# Autodesk Inventor assembly: spool holder
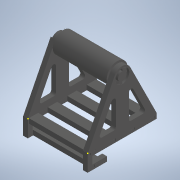
[picture p0: Inventor's stored thumbnail of the model, 180x180]
Saved by Autodesk Inventor 2020.2 (Build 242310000, 310)
## iProperties
Created: 2020-02-09
Part Number: spool holder
Document SubType Name: Assembly
Designer: mulve
Mass: 535.152 g
Surface Area: 1295.84 cm^2
Volume: 411.655 cm^3
Density: 1.3 g/cm^3
Author: mulve
## Documents named in this file (12)
- C:\Users\mulve\github\cad\spool holder\spool holder.iam
- C:\Users\mulve\github\cad\spool holder\spool holder.ipt
- C:\Users\mulve\github\cad\spool holder\spool holder arm.ipt
- C:\Users\mulve\github\cad\spool holder\spool holder span.ipt
- C:\Users\mulve\github\cad\spool holder\spool axle.ipt
- C:\Users\mulve\github\cad\spool holder\spool holder arm side2.ipt
- C:\Users\mulve\github\cad\spool holder\spool holder\AIP\FEA\d58jxclds.fins
- C:\Users\mulve\github\cad\spool holder\spool holder\AIP\FEA\d58jxclds.fsat
- C:\Users\mulve\github\cad\spool holder\spool holder\AIP\FEA\d58jxclds.ftes
- C:\Users\mulve\github\cad\spool holder\spool holder\AIP\FEA\d58jxclds.fwiz
- C:\Users\mulve\github\cad\spool holder\spool holder\AIP\FEA\d58jxclnk.fmsh
- C:\Users\mulve\github\cad\spool holder\spool holder\AIP\FEA\d58jxclnl.fres
## Components (10 placed, 5 different names)
1. spool holder:1 — Mate:4, Mate:5, Flush:1, Mate:6, Mate:7, Flush:2, Mate:8, Mate:9, Flush:3, Mate:10, Mate:11, Flush:4, Mate:12, Mate:13, Flush:5, Mate:18, Flush:8, Mate:19
2. spool holder:2 — Mate:14, Mate:15, Flush:6, Mate:16, Mate:17, Flush:7
3. spool holder arm:1 — Mate:16, Mate:17, Flush:7
4. spool holder span:1 — Mate:4, Mate:5, Flush:1
5. spool holder span:2 — Mate:6, Mate:7, Flush:2, Mate:14, Mate:15, Flush:6
6. spool holder span:3 — Mate:8, Mate:9, Flush:3
7. spool holder span:4 — Mate:10, Mate:11, Flush:4
8. spool holder span:5 — Mate:12, Mate:13, Flush:5
9. spool axle:1
10. spool holder arm side2:1 — Mate:18, Flush:8, Mate:19
## Relationships (24: Mate 16, Flush 8)
- Mate:4: spool holder:1 ↔ spool holder span:1
- Mate:5: spool holder:1 ↔ spool holder span:1
- Flush:1: spool holder:1 ↔ spool holder span:1
- Mate:6: spool holder:1 ↔ spool holder span:2
- Mate:7: spool holder:1 ↔ spool holder span:2
- Flush:2: spool holder:1 ↔ spool holder span:2
- Mate:8: spool holder:1 ↔ spool holder span:3
- Mate:9: spool holder:1 ↔ spool holder span:3
- Flush:3: spool holder:1 ↔ spool holder span:3
- Mate:10: spool holder:1 ↔ spool holder span:4
- Mate:11: spool holder:1 ↔ spool holder span:4
- Flush:4: spool holder:1 ↔ spool holder span:4
- Mate:12: spool holder:1 ↔ spool holder span:5
- Mate:13: spool holder:1 ↔ spool holder span:5
- Flush:5: spool holder:1 ↔ spool holder span:5
- Mate:14: spool holder:2 ↔ spool holder span:2
- Mate:15: spool holder:2 ↔ spool holder span:2
- Flush:6: spool holder:2 ↔ spool holder span:2
- Mate:16: spool holder:2 ↔ spool holder arm:1
- Mate:17: spool holder:2 ↔ spool holder arm:1
- Flush:7: spool holder:2 ↔ spool holder arm:1
- Mate:18: spool holder:1 ↔ spool holder arm side2:1
- Flush:8: spool holder:1 ↔ spool holder arm side2:1
- Mate:19: spool holder:1 ↔ spool holder arm side2:1
